# Autodesk Inventor assembly: WormGear5Assembly
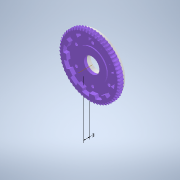
[picture p0: Inventor's stored thumbnail of the model, 180x180]
Saved by Autodesk Inventor 2022.1 (Build 261234000, 234)
## iProperties
Created: 2021-07-22
Part Number: WormGear5Assembly
Document SubType Name: Assembly
Designer: robst
Author: robst
## Documents named in this file (3)
- C:\git\CAD-Development\robSteele\ShapeWays\TelescopeProjects\TelescopeMount\forkMountForDecTripV01\Design Accelerator\WormGear5Assembly.iam
- C:\git\CAD-Development\robSteele\ShapeWays\TelescopeProjects\TelescopeMount\forkMountForDecTripV01\Design Accelerator\Worm Gear5-Bottom.ipt
- C:\git\CAD-Development\robSteele\ShapeWays\TelescopeProjects\TelescopeMount\forkMountForDecTripV01\Design Accelerator\Worm Gear5-Top.ipt
## Components (2 placed, 2 different names)
1. Worm Gear5-Bottom:1 — Insert:1, Insert:2
2. Worm Gear:1 — Insert:1, Insert:2
## Relationships (2: Insert 2)
- Insert:1: Worm Gear5-Bottom:1 ↔ Worm Gear:1
- Insert:2: Worm Gear5-Bottom:1 ↔ Worm Gear:1
